# Autodesk Inventor assembly: робот
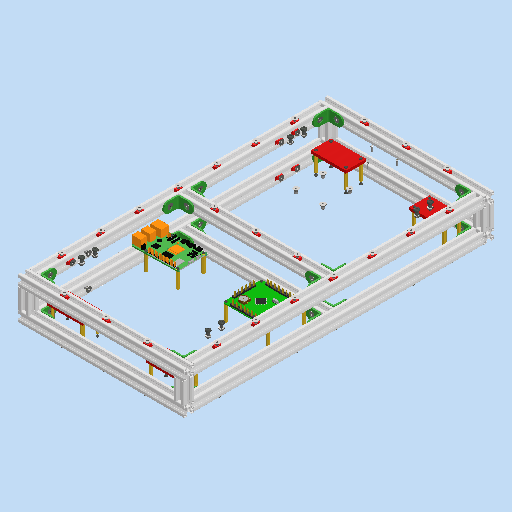
[picture p0: Inventor's stored thumbnail of the model, 512x512]
Saved by Autodesk Inventor 2025 (Build 290162000, 162)
## iProperties
Created: 2025-02-17
Part Number: робот
Document SubType Name: Assembly
Designer: volko
Mass: 11118.9 g
Surface Area: 27959 cm^2
Volume: 6182.29 cm^3
Density: 1.7985 g/cm^3
Author: volko
## Documents named in this file (62)
- C:\Users\volko\Desktop\диплом\Модели\детали\робот.iam
- C:\Users\volko\Desktop\диплом\Модели\детали\нижняя плита.ipt
- C:\Users\volko\Desktop\диплом\Модели\детали\правый привод.iam
- C:\Users\volko\Desktop\диплом\Модели\детали\левый привод.iam
- C:\Users\volko\Desktop\диплом\Модели\детали\рама.iam
- C:\Users\volko\Desktop\диплом\Модели\детали\верхняя плита.ipt
- C:\Users\volko\Desktop\диплом\Модели\детали\правый привод_MIR1.iam
- C:\Users\volko\Desktop\диплом\Модели\детали\левый привод_MIR1.iam
- C:\Users\volko\Desktop\диплом\Модели\детали\лидар.iam
- C:\Users\volko\Desktop\диплом\Модели\детали\сборка акб.iam
- C:\Users\volko\Desktop\диплом\Модели\детали\передний кожух.ipt
- C:\Users\volko\Desktop\диплом\Модели\детали\боковой кожух.ipt
- C:\Users\volko\Desktop\диплом\Модели\детали\гайка T-паза m5.ipt
- гайка T-паза m5.ipt
- C:\Users\volko\Desktop\диплом\Модели\детали\гайка T-паза m5_MIR.ipt
- C:\Users\volko\Desktop\диплом\Модели\детали\гайка T-паза m5_MIR_MIR.ipt
- C:\Users\volko\Desktop\диплом\Модели\детали\гайка T-паза m5_MIR1.ipt
- C:\Users\volko\Desktop\диплом\Модели\детали\гайка T-паза m5_MIR2.ipt
- C:\Users\volko\Desktop\диплом\Модели\детали\гайка T-паза m5_MIR_MIR1.ipt
- C:\Users\volko\Desktop\диплом\Модели\детали\лоток для маркеров.ipt
- C:\Users\volko\Desktop\диплом\Модели\детали\стандартные изделия\ru-RU\ISO 1580\ISO 1580 - M2 x 8_.ipt
- C:\Users\volko\Desktop\диплом\Модели\детали\сборка драйверов.iam
- C:\Users\volko\Desktop\диплом\Модели\детали\стандартные изделия\ru-RU\ISO 7045  H\ISO 7045 - M2,5 x 8_ - 4.8 - H - ISO.ipt
- C:\Users\volko\Desktop\диплом\Модели\детали\сборка драйверов_MIR2.iam
- C:\Users\volko\Desktop\диплом\Модели\детали\сборка драйверов_MIR3.iam
- C:\Users\volko\Desktop\диплом\Модели\детали\сборка драйверов_MIR2_MIR.iam
- C:\Users\volko\Desktop\диплом\Модели\детали\сборка raspberry pi.iam
- C:\Users\volko\Desktop\диплом\Модели\детали\сборка микроконтроллера.iam
- C:\Users\volko\Desktop\диплом\Модели\детали\стандартные изделия\ru-RU\DIN 7991(2)\DIN 7991 - M5x8.ipt
- C:\Users\volko\Desktop\диплом\Модели\детали\стандартные изделия\ru-RU\ISO 4035(2)\ISO 4035 - M5 - ISO.ipt
- C:\Users\volko\Desktop\диплом\Модели\детали\стандартные изделия\ru-RU\ISO 7380-1\ISO 7380-1 - M5 x 12.ipt
- C:\Users\volko\Desktop\диплом\Модели\детали\скоба.ipt
- C:\Users\volko\Desktop\диплом\Модели\детали\скоба_MIR.ipt
- C:\Users\volko\Desktop\диплом\Модели\детали\гайка T-паза m5_MIR_MIR1_MIR.ipt
- C:\Users\volko\Desktop\диплом\Модели\детали\скоба_MIR1.ipt
- C:\Users\volko\Desktop\диплом\Модели\детали\гайка T-паза m5_MIR_MIR1_MIR1.ipt
- C:\Users\volko\Desktop\диплом\Модели\детали\скоба_MIR_MIR.ipt
- C:\Users\volko\Desktop\диплом\Модели\детали\гайка T-паза m5_MIR_MIR1_MIR_MIR.ipt
- C:\Users\volko\Desktop\диплом\Модели\детали\скоба_MIR_MIR_MIR.ipt
- C:\Users\volko\Desktop\диплом\Модели\детали\гайка T-паза m5_MIR_MIR1_MIR_MIR_MIR.ipt
- C:\Users\volko\Desktop\диплом\Модели\детали\гайка T-паза m5_MIR_MIR1_MIR1_MIR.ipt
- C:\Users\volko\Desktop\диплом\Модели\детали\скоба_MIR1_MIR.ipt
- C:\Users\volko\Desktop\диплом\Модели\детали\скоба_MIR_MIR_MIR_MIR.ipt
- C:\Users\volko\Desktop\диплом\Модели\детали\гайка T-паза m5_MIR_MIR1_MIR_MIR_MIR_MIR.ipt
- C:\Users\volko\Desktop\диплом\Модели\детали\гайка T-паза m5_MIR_MIR1_MIR1_MIR_MIR.ipt
- C:\Users\volko\Desktop\диплом\Модели\детали\скоба_MIR1_MIR_MIR.ipt
- C:\Users\volko\Desktop\диплом\Модели\детали\скоба_MIR1_MIR_MIR_MIR.ipt
- C:\Users\volko\Desktop\диплом\Модели\детали\гайка T-паза m5_MIR_MIR1_MIR1_MIR_MIR_MIR.ipt
- C:\Users\volko\Desktop\диплом\Модели\детали\гайка T-паза m5_MIR_MIR1_MIR_MIR_MIR_MIR_MIR.ipt
- C:\Users\volko\Desktop\диплом\Модели\детали\скоба_MIR_MIR_MIR_MIR_MIR.ipt
- C:\Users\volko\Desktop\диплом\Модели\детали\скоба_MIR1_MIR_MIR1.ipt
- C:\Users\volko\Desktop\диплом\Модели\детали\гайка T-паза m5_MIR_MIR1_MIR1_MIR_MIR1.ipt
- C:\Users\volko\Desktop\диплом\Модели\детали\гайка T-паза m5_MIR_MIR1_MIR_MIR_MIR_MIR1.ipt
- C:\Users\volko\Desktop\диплом\Модели\детали\скоба_MIR_MIR_MIR_MIR1.ipt
- C:\Users\volko\Desktop\диплом\Модели\детали\скоба_MIR_MIR_MIR1.ipt
- C:\Users\volko\Desktop\диплом\Модели\детали\гайка T-паза m5_MIR_MIR1_MIR_MIR_MIR1.ipt
- C:\Users\volko\Desktop\диплом\Модели\детали\гайка T-паза m5_MIR_MIR1_MIR1_MIR1.ipt
- C:\Users\volko\Desktop\диплом\Модели\детали\скоба_MIR1_MIR1.ipt
- C:\Users\volko\Desktop\диплом\Модели\детали\гайка T-паза m5_MIR_MIR1_MIR_MIR2.ipt
- C:\Users\volko\Desktop\диплом\Модели\детали\скоба_MIR_MIR2.ipt
- C:\Users\volko\Desktop\диплом\Модели\детали\скоба_MIR4.ipt
- C:\Users\volko\Desktop\диплом\Модели\детали\гайка T-паза m5_MIR_MIR1_MIR3.ipt
## Components (261 placed, 60 different names)
1. рама:1 [sub-assembly] — Совмещение:1, Совмещение:3, Совмещение:4, Совмещение:12, Совмещение:13, Совмещение:15, Совмещение:16, Совмещение:18, Совмещение:19, Совмещение:20, Заподлицо:19, Заподлицо:20, Совмещение:23, Заподлицо:22, Совмещение:25, Совмещение:26, Совмещение:27, Совмещение:28, Совмещение:29, Совмещение:32, Совмещение:38, Угол:2, Совмещение:40, Угол:3, Заподлицо:60, Совмещение:88, Совмещение:89, Заподлицо:69
2. правый привод:1 [sub-assembly] — Совмещение:11, Заподлицо:10, Совмещение:12, Совмещение:80, Совмещение:81
3. левый привод:1 [sub-assembly] — Совмещение:3, Совмещение:4, Заподлицо:2, Совмещение:11, Заподлицо:10, Совмещение:13
4. правый привод_MIR1:1 [sub-assembly] — Заподлицо:12, Совмещение:14, Совмещение:19, Совмещение:21
5. левый привод_MIR1:1 [sub-assembly] — Заподлицо:12, Совмещение:14, Совмещение:15, Совмещение:20, Совмещение:33, Совмещение:34, Совмещение:35, Совмещение:36, Совмещение:37
6. нижняя плита:1 — Заподлицо:14, Совмещение:16, Заподлицо:21, Совмещение:25, Заподлицо:27, Заподлицо:30, Заподлицо:31, Заподлицо:32, Совмещение:41, Совмещение:42, Совмещение:43, Совмещение:44, Заподлицо:35, Совмещение:58, Совмещение:59, Совмещение:60, Совмещение:61, Совмещение:62, Совмещение:63, Совмещение:64, Совмещение:65, Совмещение:66, Совмещение:67, Совмещение:72, Совмещение:73
7. верхняя плита:1 — Совмещение:17, Совмещение:18, Заподлицо:22, Совмещение:24, Совмещение:48, Совмещение:49, Совмещение:50, Совмещение:51, Заподлицо:37, Заподлицо:38, Заподлицо:39, Заподлицо:40, Заподлицо:41, Заподлицо:42, Заподлицо:43, Заподлицо:44, Заподлицо:45, Заподлицо:46, Заподлицо:47, Заподлицо:48, Заподлицо:49, Заподлицо:50, Заподлицо:51, Заподлицо:52, Заподлицо:53, Заподлицо:54, Заподлицо:55, Заподлицо:56, Заподлицо:57, Заподлицо:58, Заподлицо:59, Совмещение:74, Совмещение:75, Совмещение:76, Совмещение:77
8. лидар:1 [sub-assembly] — Совмещение:24, Заподлицо:26, Совмещение:51, Совмещение:52, Совмещение:53, Совмещение:54, Совмещение:55, Совмещение:56, Совмещение:57
9. сборка акб:1 [sub-assembly] — Заподлицо:21, Совмещение:22, Совмещение:23
10. передний кожух:1 — Совмещение:26, Заподлицо:27, Заподлицо:33
11. передний кожух:2 — Совмещение:27, Заподлицо:30, Заподлицо:34
12. боковой кожух:1 — Совмещение:28, Заподлицо:31, Совмещение:30
13. боковой кожух:2 — Совмещение:29, Заподлицо:32, Совмещение:31
14. лоток для маркеров:1 — Совмещение:47, Совмещение:48, Совмещение:49, Заподлицо:36
15. сборка драйверов:1 [sub-assembly] — Совмещение:58, Совмещение:59, Совмещение:68
16. сборка драйверов_MIR2:1 [sub-assembly] — Совмещение:69
17. сборка драйверов_MIR3:1 [sub-assembly] — Совмещение:70
18. сборка драйверов_MIR2_MIR:1 [sub-assembly] — Совмещение:71
19. сборка raspberry pi:1 [sub-assembly] — Совмещение:72
20. сборка микроконтроллера:1 [sub-assembly] — Совмещение:73
21. скоба_MIR1_MIR_MIR_MIR:1 — Совмещение:180, Совмещение:181, Угол:38, Совмещение:182, Совмещение:183, Угол:39, Заподлицо:96, Заподлицо:97
22. гайка T-паза m5_MIR_MIR1_MIR1_MIR_MIR_MIR:1 — Совмещение:180, Совмещение:181, Угол:38
23. гайка T-паза m5_MIR_MIR1_MIR1_MIR_MIR_MIR:2 — Совмещение:182, Совмещение:183, Угол:39
24. DIN 7991 M5x8:95 — Заподлицо:96
25. DIN 7991 M5x8:96 — Заподлицо:97
26. гайка T-паза m5_MIR_MIR1_MIR_MIR_MIR_MIR_MIR:1 — Угол:37, Совмещение:178, Совмещение:179
27. гайка T-паза m5_MIR_MIR1_MIR_MIR_MIR_MIR_MIR:2 — Угол:36, Совмещение:175, Совмещение:176, Совмещение:177
28. скоба_MIR_MIR_MIR_MIR_MIR:1 — Заподлицо:94, Совмещение:174, Заподлицо:95, Угол:36, Совмещение:175, Совмещение:176, Угол:37, Совмещение:178, Совмещение:179
29. DIN 7991 M5x8:97 — Заподлицо:95, Совмещение:177
30. DIN 7991 M5x8:98 — Заподлицо:94, Совмещение:174
31. скоба_MIR1_MIR_MIR1:1 — Заподлицо:92, Заподлицо:93, Угол:34, Совмещение:170, Совмещение:171, Угол:35, Совмещение:172, Совмещение:173
32. гайка T-паза m5_MIR_MIR1_MIR1_MIR_MIR1:1 — Угол:35, Совмещение:172, Совмещение:173
33. гайка T-паза m5_MIR_MIR1_MIR1_MIR_MIR1:2 — Угол:34, Совмещение:170, Совмещение:171
34. DIN 7991 M5x8:99 — Заподлицо:93
35. DIN 7991 M5x8:100 — Заподлицо:92
36. гайка T-паза m5_MIR_MIR1_MIR_MIR_MIR_MIR1:1 — Совмещение:168, Совмещение:169, Угол:33
37. гайка T-паза m5_MIR_MIR1_MIR_MIR_MIR_MIR1:2 — Совмещение:165, Совмещение:166, Совмещение:167, Угол:32
38. скоба_MIR_MIR_MIR_MIR1:1 — Заподлицо:90, Совмещение:164, Заподлицо:91, Совмещение:166, Совмещение:167, Угол:32, Совмещение:168, Совмещение:169, Угол:33
39. DIN 7991 M5x8:101 — Заподлицо:90, Совмещение:165
40. DIN 7991 M5x8:102 — Совмещение:164, Заподлицо:91
41. скоба_MIR_MIR_MIR1:1 — Угол:30, Совмещение:158, Совмещение:159, Угол:31, Совмещение:160, Совмещение:161, Заподлицо:88, Совмещение:162, Заподлицо:89
42. DIN 7991 M5x8:103 — Совмещение:163, Заподлицо:89
43. DIN 7991 M5x8:104 — Заподлицо:88, Совмещение:162
44. гайка T-паза m5_MIR_MIR1_MIR_MIR_MIR1:1 — Угол:31, Совмещение:160, Совмещение:161, Совмещение:163
45. гайка T-паза m5_MIR_MIR1_MIR_MIR_MIR1:2 — Угол:30, Совмещение:158, Совмещение:159
46. DIN 7991 M5x8:105 — Заподлицо:87
47. DIN 7991 M5x8:106 — Заподлицо:86
48. гайка T-паза m5_MIR_MIR1_MIR1_MIR1:1 — Совмещение:156, Совмещение:157, Угол:29
49. гайка T-паза m5_MIR_MIR1_MIR1_MIR1:2 — Совмещение:154, Совмещение:155, Угол:28
50. скоба_MIR1_MIR1:1 — Совмещение:154, Совмещение:155, Угол:28, Совмещение:156, Совмещение:157, Угол:29, Заподлицо:86, Заподлицо:87
51. DIN 7991 M5x8:107 — Заподлицо:85
52. DIN 7991 M5x8:108 — Заподлицо:84
53. гайка T-паза m5_MIR_MIR1_MIR_MIR2:1 — Совмещение:152, Совмещение:153, Угол:27
54. гайка T-паза m5_MIR_MIR1_MIR_MIR2:2 — Совмещение:150, Совмещение:151, Угол:26
55. скоба_MIR_MIR2:1 — Совмещение:150, Совмещение:151, Угол:26, Совмещение:152, Совмещение:153, Угол:27, Заподлицо:84, Заподлицо:85
56. скоба_MIR4:1 — Угол:24, Совмещение:144, Совмещение:145, Угол:25, Совмещение:146, Совмещение:147, Заподлицо:82, Совмещение:148, Заподлицо:83
57. гайка T-паза m5_MIR_MIR1_MIR3:1 — Угол:24, Совмещение:144, Совмещение:145
58. гайка T-паза m5_MIR_MIR1_MIR3:2 — Угол:25, Совмещение:146, Совмещение:147, Совмещение:149
59. DIN 7991 M5x8:109 — Заподлицо:82, Совмещение:148
60. DIN 7991 M5x8:110 — Совмещение:149, Заподлицо:83
61. ISO 7380-1 M5 x 12:8 — Совмещение:87
62. ISO 7380-1 M5 x 12:7 — Совмещение:86
63. ISO 4035 M5:8 — Совмещение:87
64. ISO 4035 M5:7 — Совмещение:86
65. ISO 7380-1 M5 x 12:6 — Совмещение:85
66. ISO 7380-1 M5 x 12:5 — Совмещение:84
67. ISO 4035 M5:6 — Совмещение:85
68. ISO 4035 M5:5 — Совмещение:84
69. ISO 7380-1 M5 x 12:4 — Совмещение:83
70. ISO 7380-1 M5 x 12:3 — Совмещение:82
71. ISO 4035 M5:4 — Совмещение:83
72. ISO 4035 M5:3 — Совмещение:82
73. ISO 7380-1 M5 x 12:2 — Совмещение:75, Совмещение:77, Совмещение:79
74. ISO 7380-1 M5 x 12:1 — Совмещение:74, Совмещение:76, Совмещение:78
75. ISO 4035 M5:2 — Совмещение:79, Совмещение:81
76. ISO 4035 M5:1 — Совмещение:78, Совмещение:80
77. DIN 7991 M5x8:74
78. DIN 7991 M5x8:73
79. DIN 7991 M5x8:72
80. DIN 7991 M5x8:71
81. DIN 7991 M5x8:78
82. DIN 7991 M5x8:77
83. DIN 7991 M5x8:76
84. DIN 7991 M5x8:75
85. DIN 7991 M5x8:70
86. DIN 7991 M5x8:69
87. DIN 7991 M5x8:68
88. DIN 7991 M5x8:67
89. ISO 7045 H M2,5 x 8 - 4.8 - H:5
90. ISO 7045 H M2,5 x 8 - 4.8 - H:6
91. ISO 7045 H M2,5 x 8 - 4.8 - H:7
92. ISO 7045 H M2,5 x 8 - 4.8 - H:8 — Совмещение:69
93. ISO 7045 H M2,5 x 8 - 4.8 - H:9
94. ISO 7045 H M2,5 x 8 - 4.8 - H:10
95. ISO 7045 H M2,5 x 8 - 4.8 - H:11
96. ISO 7045 H M2,5 x 8 - 4.8 - H:12 — Совмещение:70
97. ISO 7045 H M2,5 x 8 - 4.8 - H:13
98. ISO 7045 H M2,5 x 8 - 4.8 - H:14
99. ISO 7045 H M2,5 x 8 - 4.8 - H:15
100. ISO 7045 H M2,5 x 8 - 4.8 - H:16 — Совмещение:71
101. ISO 7045 H M2,5 x 8 - 4.8 - H:1 — Совмещение:60, Совмещение:66
102. ISO 7045 H M2,5 x 8 - 4.8 - H:2 — Совмещение:63, Совмещение:65
103. ISO 7045 H M2,5 x 8 - 4.8 - H:3 — Совмещение:62, Совмещение:64
104. ISO 7045 H M2,5 x 8 - 4.8 - H:4 — Совмещение:61, Совмещение:67, Совмещение:68
105. ISO 1580 M2 x 8:3 — Совмещение:54, Совмещение:55
106. ISO 1580 M2 x 8:2 — Совмещение:53, Совмещение:57
107. ISO 1580 M2 x 8:1 — Совмещение:52, Совмещение:56
108. гайка T-паза m5_MIR_MIR1:10
109. гайка T-паза m5_MIR_MIR1:11
110. гайка T-паза m5_MIR_MIR1:13
111. гайка T-паза m5_MIR_MIR1:12
112. гайка T-паза m5_MIR_MIR1:14
113. DIN 7991 M5x8:2 — Заподлицо:37
114. DIN 7991 M5x8:3 — Заподлицо:56
115. DIN 7991 M5x8:4 — Заподлицо:47
116. DIN 7991 M5x8:5 — Заподлицо:38
117. DIN 7991 M5x8:6 — Заподлицо:55
118. DIN 7991 M5x8:7 — Заподлицо:48
119. DIN 7991 M5x8:8 — Заподлицо:40
120. DIN 7991 M5x8:9 — Заподлицо:54
121. DIN 7991 M5x8:10 — Заподлицо:49
122. DIN 7991 M5x8:11 — Совмещение:46, Заподлицо:39
123. DIN 7991 M5x8:12 — Заподлицо:59
124. DIN 7991 M5x8:13 — Заподлицо:41
125. DIN 7991 M5x8:14 — Заподлицо:58
126. DIN 7991 M5x8:15 — Заподлицо:42
127. DIN 7991 M5x8:16 — Заподлицо:57
128. DIN 7991 M5x8:17 — Заподлицо:43
129. DIN 7991 M5x8:18 — Заподлицо:53
130. DIN 7991 M5x8:19 — Заподлицо:44
131. DIN 7991 M5x8:20 — Заподлицо:52
132. DIN 7991 M5x8:21 — Заподлицо:45
133. DIN 7991 M5x8:22 — Заподлицо:51
134. DIN 7991 M5x8:23 — Заподлицо:46
135. DIN 7991 M5x8:24 — Заподлицо:50
136. гайка T-паза m5_MIR2:7
137. гайка T-паза m5_MIR2:6
138. гайка T-паза m5_MIR2:5
139. гайка T-паза m5_MIR2:2
140. гайка T-паза m5_MIR2:1
141. гайка T-паза m5_MIR2:4
142. гайка T-паза m5_MIR2:3
143. гайка T-паза m5_MIR2:8
144. гайка T-паза m5_MIR2:9
145. гайка T-паза m5_MIR_MIR1:1 — Совмещение:46
146. гайка T-паза m5_MIR_MIR1:2
147. гайка T-паза m5_MIR_MIR1:3
148. гайка T-паза m5_MIR_MIR1:4
149. гайка T-паза m5_MIR_MIR1:6
150. гайка T-паза m5_MIR_MIR1:5
151. гайка T-паза m5_MIR_MIR1:7
152. гайка T-паза m5_MIR_MIR1:8
153. гайка T-паза m5_MIR_MIR1:9
154. гайка T-паза m5_MIR1:4
155. гайка T-паза m5_MIR1:3
156. гайка T-паза m5_MIR1:2
157. гайка T-паза m5_MIR1:1
158. гайка T-паза m5_MIR_MIR:4
159. гайка T-паза m5_MIR_MIR:3
160. гайка T-паза m5_MIR_MIR:2
161. гайка T-паза m5_MIR_MIR:1
162. гайка T-паза m5_MIR:4
163. гайка T-паза m5_MIR:3
164. гайка T-паза m5_MIR:2
165. гайка T-паза m5_MIR:1
166. DIN 7991 M5x8:37 — Совмещение:34
167. DIN 7991 M5x8:38 — Совмещение:35
168. DIN 7991 M5x8:39 — Совмещение:36
169. DIN 7991 M5x8:1 — Совмещение:37
170. скоба_MIR1_MIR_MIR:1 — Заподлицо:80, Заподлицо:81, Угол:22, Совмещение:140, Совмещение:141, Угол:23, Совмещение:142, Совмещение:143
171. гайка T-паза m5_MIR_MIR1_MIR1_MIR_MIR:2 — Угол:23, Совмещение:142, Совмещение:143
172. гайка T-паза m5_MIR_MIR1_MIR1_MIR_MIR:1 — Угол:22, Совмещение:140, Совмещение:141
173. DIN 7991 M5x8:94 — Заподлицо:81
174. DIN 7991 M5x8:93 — Заподлицо:80
175. гайка T-паза m5_MIR_MIR1_MIR_MIR_MIR_MIR:2 — Совмещение:138, Совмещение:139, Угол:21
176. гайка T-паза m5_MIR_MIR1_MIR_MIR_MIR_MIR:1 — Совмещение:135, Совмещение:136, Совмещение:137, Угол:20
177. скоба_MIR_MIR_MIR_MIR:1 — Заподлицо:78, Совмещение:134, Заподлицо:79, Совмещение:136, Совмещение:137, Угол:20, Совмещение:138, Совмещение:139, Угол:21
178. DIN 7991 M5x8:92 — Заподлицо:78, Совмещение:135
179. DIN 7991 M5x8:91 — Совмещение:134, Заподлицо:79
180. скоба_MIR1_MIR:1 — Совмещение:124, Совмещение:125, Угол:16, Совмещение:126, Совмещение:127, Угол:17, Заподлицо:74, Заподлицо:75
181. гайка T-паза m5_MIR_MIR1_MIR1_MIR:2 — Совмещение:124, Совмещение:125, Угол:16
182. гайка T-паза m5_MIR_MIR1_MIR1_MIR:1 — Совмещение:126, Совмещение:127, Угол:17
183. DIN 7991 M5x8:90 — Заподлицо:74
184. DIN 7991 M5x8:89 — Заподлицо:75
185. гайка T-паза m5_MIR_MIR1_MIR_MIR_MIR:2 — Угол:18, Совмещение:128, Совмещение:129
186. гайка T-паза m5_MIR_MIR1_MIR_MIR_MIR:1 — Угол:19, Совмещение:130, Совмещение:131, Совмещение:133
187. скоба_MIR_MIR_MIR:1 — Угол:18, Совмещение:128, Совмещение:129, Угол:19, Совмещение:130, Совмещение:131, Заподлицо:76, Совмещение:132, Заподлицо:77
188. DIN 7991 M5x8:87 — Совмещение:133, Заподлицо:77
189. DIN 7991 M5x8:88 — Заподлицо:76, Совмещение:132
190. скоба_MIR_MIR:1 — Совмещение:108, Совмещение:109, Угол:10, Совмещение:110, Совмещение:111, Угол:11, Совмещение:112, Заподлицо:67, Заподлицо:68
191. DIN 7991 M5x8:86 — Заподлицо:68, Совмещение:113
192. DIN 7991 M5x8:85 — Совмещение:112, Заподлицо:67
193. гайка T-паза m5_MIR_MIR1_MIR_MIR:2 — Совмещение:110, Совмещение:111, Угол:11, Совмещение:113
194. гайка T-паза m5_MIR_MIR1_MIR_MIR:1 — Совмещение:108, Совмещение:109, Угол:10
195. DIN 7991 M5x8:84 — Заподлицо:66
196. DIN 7991 M5x8:83 — Заподлицо:65
197. гайка T-паза m5_MIR_MIR1_MIR1:2 — Угол:9, Совмещение:104, Совмещение:105
198. гайка T-паза m5_MIR_MIR1_MIR1:1 — Угол:8, Совмещение:102, Совмещение:103
199. скоба_MIR1:1 — Угол:8, Совмещение:102, Совмещение:103, Угол:9, Совмещение:104, Совмещение:105, Заподлицо:65, Заподлицо:66
200. DIN 7991 M5x8:82 — Заподлицо:64
201. DIN 7991 M5x8:81 — Заподлицо:63
202. гайка T-паза m5_MIR_MIR1_MIR:2 — Угол:7, Совмещение:98, Совмещение:99
203. гайка T-паза m5_MIR_MIR1_MIR:1 — Угол:6, Совмещение:96, Совмещение:97
204. скоба_MIR:1 — Угол:6, Совмещение:96, Совмещение:97, Угол:7, Совмещение:98, Совмещение:99, Заподлицо:63, Заподлицо:64
205. скоба:1 — Заподлицо:60, Совмещение:88, Совмещение:89, Совмещение:90, Совмещение:91, Совмещение:92, Совмещение:93, Угол:4, Угол:5, Совмещение:94, Заподлицо:61, Заподлицо:62
206. гайка T-паза m5_MIR_MIR1:15 — Совмещение:90, Совмещение:92, Угол:4
207. гайка T-паза m5_MIR_MIR1:16 — Совмещение:91, Совмещение:93, Угол:5, Совмещение:95
208. DIN 7991 M5x8:79 — Совмещение:94, Заподлицо:61
209. DIN 7991 M5x8:80 — Заподлицо:62, Совмещение:95
210. DIN 7991 M5x8:63 — Совмещение:50, Заподлицо:36
211. DIN 7991 M5x8:64
212. DIN 7991 M5x8:65
213. DIN 7991 M5x8:66
214. DIN 7991 M5x8:49 — Совмещение:45, Заподлицо:35
215. DIN 7991 M5x8:50
216. DIN 7991 M5x8:51
217. DIN 7991 M5x8:52
218. DIN 7991 M5x8:53
219. DIN 7991 M5x8:54
220. DIN 7991 M5x8:55
221. DIN 7991 M5x8:56
222. DIN 7991 M5x8:57
223. DIN 7991 M5x8:58
224. DIN 7991 M5x8:59
225. DIN 7991 M5x8:60
226. DIN 7991 M5x8:61
227. DIN 7991 M5x8:62
228. гайка T-паза m5_MIR:5 — Совмещение:40, Угол:3, Совмещение:42, Совмещение:45
229. гайка T-паза m5_MIR:6
230. гайка T-паза m5_MIR:7
231. гайка T-паза m5_MIR:8
232. гайка T-паза m5_MIR:9
233. гайка T-паза m5_MIR:10
234. гайка T-паза m5_MIR:11
235. гайка T-паза m5_MIR:12
236. гайка T-паза m5_MIR:13
237. гайка T-паза m5_MIR:14
238. гайка T-паза m5_MIR:15
239. гайка T-паза m5_MIR:16
240. гайка T-паза m5_MIR:17
241. гайка T-паза m5_MIR:18
242. DIN 7991 M5x8:40 — Совмещение:43, Совмещение:44
243. DIN 7991 M5x8:41
244. DIN 7991 M5x8:42
245. DIN 7991 M5x8:43
246. DIN 7991 M5x8:44
247. DIN 7991 M5x8:45
248. DIN 7991 M5x8:46
249. DIN 7991 M5x8:47
250. DIN 7991 M5x8:48
251. гайка T-паза m5:5 — Совмещение:38, Угол:2, Совмещение:41
252. гайка T-паза m5:6
253. гайка T-паза m5:7
254. гайка T-паза m5:8
255. гайка T-паза m5:9
256. гайка T-паза m5:10
257. гайка T-паза m5:11
258. гайка T-паза m5:12
259. гайка T-паза m5:13
260. гайка T-паза m5:1 — Совмещение:32, Совмещение:33, Угол:1
261. гайка T-паза m5:2
## Component patterns: (4 elements, first: DIN 7991 M5x8:63), (14 elements, first: DIN 7991 M5x8:49), (14 elements, first: гайка T-паза m5_MIR:5), (9 elements, first: DIN 7991 M5x8:40), (9 elements, first: гайка T-паза m5:5), (2 elements, first: гайка T-паза m5:1)
## Relationships (271: Mate 161, Flush 75, Angle 35)
- Совмещение:1 [Mate]: рама:1
- Совмещение:3 [Mate]: рама:1 ↔ левый привод:1
- Совмещение:4 [Mate]: рама:1 ↔ левый привод:1
- Заподлицо:2 [Flush]: левый привод:1
- Совмещение:11 [Mate]: правый привод:1 ↔ левый привод:1
- Заподлицо:10 [Flush]: правый привод:1 ↔ левый привод:1
- Совмещение:12 [Mate]: рама:1 ↔ правый привод:1
- Совмещение:13 [Mate] (50 mm): рама:1 ↔ левый привод:1
- Заподлицо:12 [Flush]: правый привод_MIR1:1 ↔ левый привод_MIR1:1
- Совмещение:14 [Mate]: правый привод_MIR1:1 ↔ левый привод_MIR1:1
- Совмещение:15 [Mate] (50 mm): рама:1 ↔ левый привод_MIR1:1
- Заподлицо:14 [Flush]: нижняя плита:1
- Совмещение:16 [Mate]: рама:1 ↔ нижняя плита:1
- Совмещение:17 [Mate]: верхняя плита:1
- Совмещение:18 [Mate]: рама:1 ↔ верхняя плита:1
- Совмещение:19 [Mate]: рама:1 ↔ правый привод_MIR1:1
- Совмещение:20 [Mate]: рама:1 ↔ левый привод_MIR1:1
- Заподлицо:18 [Flush]
- Заподлицо:19 [Flush]: рама:1
- Заподлицо:20 [Flush]: рама:1
- Совмещение:21 [Mate]: правый привод_MIR1:1
- Заподлицо:21 [Flush]: нижняя плита:1 ↔ сборка акб:1
- Совмещение:22 [Mate]: сборка акб:1
- Совмещение:23 [Mate] (10 mm): рама:1 ↔ сборка акб:1
- Заподлицо:22 [Flush]: рама:1 ↔ верхняя плита:1
- Совмещение:24 [Mate]: верхняя плита:1 ↔ лидар:1
- Заподлицо:26 [Flush]: лидар:1
- Совмещение:25 [Mate]: рама:1 ↔ нижняя плита:1
- Совмещение:26 [Mate]: рама:1 ↔ передний кожух:1
- Заподлицо:27 [Flush]: нижняя плита:1 ↔ передний кожух:1
- Совмещение:27 [Mate]: рама:1 ↔ передний кожух:2
- Заподлицо:30 [Flush]: нижняя плита:1 ↔ передний кожух:2
- Совмещение:28 [Mate]: рама:1 ↔ боковой кожух:1
- Совмещение:29 [Mate]: рама:1 ↔ боковой кожух:2
- Заподлицо:31 [Flush]: нижняя плита:1 ↔ боковой кожух:1
- Заподлицо:32 [Flush]: нижняя плита:1 ↔ боковой кожух:2
- Заподлицо:33 [Flush]: передний кожух:1
- Заподлицо:34 [Flush]: передний кожух:2
- Совмещение:30 [Mate]: боковой кожух:1
- Совмещение:31 [Mate]: боковой кожух:2
- Совмещение:32 [Mate]: рама:1 ↔ гайка T-паза m5:1
- Совмещение:33 [Mate]: левый привод_MIR1:1 ↔ гайка T-паза m5:1
- Угол:1 [Angle] (0 deg): гайка T-паза m5:1
- Совмещение:34 [Mate]: левый привод_MIR1:1 ↔ DIN 7991 M5x8:37
- Совмещение:35 [Mate]: левый привод_MIR1:1 ↔ DIN 7991 M5x8:38
- Совмещение:36 [Mate]: левый привод_MIR1:1 ↔ DIN 7991 M5x8:39
- Совмещение:37 [Mate]: левый привод_MIR1:1 ↔ DIN 7991 M5x8:1
- Совмещение:38 [Mate]: рама:1 ↔ гайка T-паза m5:5
- Угол:2 [Angle] (0 deg): рама:1 ↔ гайка T-паза m5:5
- Совмещение:40 [Mate]: рама:1 ↔ гайка T-паза m5_MIR:5
- Угол:3 [Angle] (0 deg): рама:1 ↔ гайка T-паза m5_MIR:5
- Совмещение:41 [Mate]: нижняя плита:1 ↔ гайка T-паза m5:5
- Совмещение:42 [Mate]: нижняя плита:1 ↔ гайка T-паза m5_MIR:5
- Совмещение:43 [Mate]: нижняя плита:1 ↔ DIN 7991 M5x8:40
- Совмещение:44 [Mate]: нижняя плита:1 ↔ DIN 7991 M5x8:40
- Совмещение:45 [Mate]: DIN 7991 M5x8:49 ↔ гайка T-паза m5_MIR:5
- Заподлицо:35 [Flush]: нижняя плита:1 ↔ DIN 7991 M5x8:49
- Совмещение:46 [Mate]: DIN 7991 M5x8:11 ↔ гайка T-паза m5_MIR_MIR1:1
- Совмещение:47 [Mate]: лоток для маркеров:1
- Совмещение:48 [Mate]: верхняя плита:1 ↔ лоток для маркеров:1
- Совмещение:49 [Mate]: верхняя плита:1 ↔ лоток для маркеров:1
- Совмещение:50 [Mate]: верхняя плита:1 ↔ DIN 7991 M5x8:63
- Заподлицо:36 [Flush]: лоток для маркеров:1 ↔ DIN 7991 M5x8:63
- Совмещение:51 [Mate]: верхняя плита:1 ↔ лидар:1
- Совмещение:52 [Mate]: лидар:1 ↔ ISO 1580 M2 x 8:1
- Совмещение:53 [Mate]: лидар:1 ↔ ISO 1580 M2 x 8:2
- Совмещение:54 [Mate]: лидар:1 ↔ ISO 1580 M2 x 8:3
- Совмещение:55 [Mate]: лидар:1 ↔ ISO 1580 M2 x 8:3
- Совмещение:56 [Mate]: лидар:1 ↔ ISO 1580 M2 x 8:1
- Совмещение:57 [Mate]: лидар:1 ↔ ISO 1580 M2 x 8:2
- Заподлицо:37 [Flush]: верхняя плита:1 ↔ DIN 7991 M5x8:2
- Заподлицо:38 [Flush]: верхняя плита:1 ↔ DIN 7991 M5x8:5
- Заподлицо:39 [Flush]: верхняя плита:1 ↔ DIN 7991 M5x8:11
- Заподлицо:40 [Flush]: верхняя плита:1 ↔ DIN 7991 M5x8:8
- Заподлицо:41 [Flush]: верхняя плита:1 ↔ DIN 7991 M5x8:13
- Заподлицо:42 [Flush]: верхняя плита:1 ↔ DIN 7991 M5x8:15
- Заподлицо:43 [Flush]: верхняя плита:1 ↔ DIN 7991 M5x8:17
- Заподлицо:44 [Flush]: верхняя плита:1 ↔ DIN 7991 M5x8:19
- Заподлицо:45 [Flush]: верхняя плита:1 ↔ DIN 7991 M5x8:21
- Заподлицо:46 [Flush]: верхняя плита:1 ↔ DIN 7991 M5x8:23
- Заподлицо:47 [Flush]: верхняя плита:1 ↔ DIN 7991 M5x8:4
- Заподлицо:48 [Flush]: верхняя плита:1 ↔ DIN 7991 M5x8:7
- Заподлицо:49 [Flush]: верхняя плита:1 ↔ DIN 7991 M5x8:10
- Заподлицо:50 [Flush]: верхняя плита:1 ↔ DIN 7991 M5x8:24
- Заподлицо:51 [Flush]: верхняя плита:1 ↔ DIN 7991 M5x8:22
- Заподлицо:52 [Flush]: верхняя плита:1 ↔ DIN 7991 M5x8:20
- Заподлицо:53 [Flush]: верхняя плита:1 ↔ DIN 7991 M5x8:18
- Заподлицо:54 [Flush]: верхняя плита:1 ↔ DIN 7991 M5x8:9
- Заподлицо:55 [Flush]: верхняя плита:1 ↔ DIN 7991 M5x8:6
- Заподлицо:56 [Flush]: верхняя плита:1 ↔ DIN 7991 M5x8:3
- Заподлицо:57 [Flush]: верхняя плита:1 ↔ DIN 7991 M5x8:16
- Заподлицо:58 [Flush]: верхняя плита:1 ↔ DIN 7991 M5x8:14
- Заподлицо:59 [Flush]: верхняя плита:1 ↔ DIN 7991 M5x8:12
- Совмещение:58 [Mate]: нижняя плита:1 ↔ сборка драйверов:1
- Совмещение:59 [Mate]: нижняя плита:1 ↔ сборка драйверов:1
- Совмещение:60 [Mate]: нижняя плита:1 ↔ ISO 7045 H M2,5 x 8 - 4.8 - H:1
- Совмещение:61 [Mate]: нижняя плита:1 ↔ ISO 7045 H M2,5 x 8 - 4.8 - H:4
- Совмещение:62 [Mate]: нижняя плита:1 ↔ ISO 7045 H M2,5 x 8 - 4.8 - H:3
- Совмещение:63 [Mate]: нижняя плита:1 ↔ ISO 7045 H M2,5 x 8 - 4.8 - H:2
- Совмещение:64 [Mate]: нижняя плита:1 ↔ ISO 7045 H M2,5 x 8 - 4.8 - H:3
- Совмещение:65 [Mate]: нижняя плита:1 ↔ ISO 7045 H M2,5 x 8 - 4.8 - H:2
- Совмещение:66 [Mate]: нижняя плита:1 ↔ ISO 7045 H M2,5 x 8 - 4.8 - H:1
- Совмещение:67 [Mate]: нижняя плита:1 ↔ ISO 7045 H M2,5 x 8 - 4.8 - H:4
- Совмещение:68 [Mate]: сборка драйверов:1 ↔ ISO 7045 H M2,5 x 8 - 4.8 - H:4
- Совмещение:69 [Mate]: сборка драйверов_MIR2:1 ↔ ISO 7045 H M2,5 x 8 - 4.8 - H:8
- Совмещение:70 [Mate]: сборка драйверов_MIR3:1 ↔ ISO 7045 H M2,5 x 8 - 4.8 - H:12
- Совмещение:71 [Mate]: сборка драйверов_MIR2_MIR:1 ↔ ISO 7045 H M2,5 x 8 - 4.8 - H:16
- Совмещение:72 [Mate]: нижняя плита:1 ↔ сборка raspberry pi:1
- Совмещение:73 [Mate]: нижняя плита:1 ↔ сборка микроконтроллера:1
- Совмещение:74 [Mate]: верхняя плита:1 ↔ ISO 7380-1 M5 x 12:1
- Совмещение:75 [Mate]: верхняя плита:1 ↔ ISO 7380-1 M5 x 12:2
- Совмещение:76 [Mate]: верхняя плита:1 ↔ ISO 7380-1 M5 x 12:1
- Совмещение:77 [Mate]: верхняя плита:1 ↔ ISO 7380-1 M5 x 12:2
- Совмещение:78 [Mate]: ISO 7380-1 M5 x 12:1 ↔ ISO 4035 M5:1
- Совмещение:79 [Mate]: ISO 7380-1 M5 x 12:2 ↔ ISO 4035 M5:2
- Совмещение:80 [Mate]: правый привод:1 ↔ ISO 4035 M5:1
- Совмещение:81 [Mate]: правый привод:1 ↔ ISO 4035 M5:2
- Совмещение:82 [Mate]: ISO 7380-1 M5 x 12:3 ↔ ISO 4035 M5:3
- Совмещение:83 [Mate]: ISO 7380-1 M5 x 12:4 ↔ ISO 4035 M5:4
- Совмещение:84 [Mate]: ISO 7380-1 M5 x 12:5 ↔ ISO 4035 M5:5
- Совмещение:85 [Mate]: ISO 7380-1 M5 x 12:6 ↔ ISO 4035 M5:6
- Совмещение:86 [Mate]: ISO 7380-1 M5 x 12:7 ↔ ISO 4035 M5:7
- Совмещение:87 [Mate]: ISO 7380-1 M5 x 12:8 ↔ ISO 4035 M5:8
- Заподлицо:60 [Flush]: рама:1 ↔ скоба:1
- Совмещение:88 [Mate]: рама:1 ↔ скоба:1
- Совмещение:89 [Mate]: рама:1 ↔ скоба:1
- Совмещение:90 [Mate]: скоба:1 ↔ гайка T-паза m5_MIR_MIR1:15
- Совмещение:91 [Mate]: скоба:1 ↔ гайка T-паза m5_MIR_MIR1:16
- Совмещение:92 [Mate]: скоба:1 ↔ гайка T-паза m5_MIR_MIR1:15
- Совмещение:93 [Mate]: скоба:1 ↔ гайка T-паза m5_MIR_MIR1:16
- Угол:4 [Angle] (0 deg): скоба:1 ↔ гайка T-паза m5_MIR_MIR1:15
- Угол:5 [Angle] (0 deg): скоба:1 ↔ гайка T-паза m5_MIR_MIR1:16
- Совмещение:94 [Mate]: скоба:1 ↔ DIN 7991 M5x8:79
- Заподлицо:61 [Flush]: скоба:1 ↔ DIN 7991 M5x8:79
- Заподлицо:62 [Flush]: скоба:1 ↔ DIN 7991 M5x8:80
- Совмещение:95 [Mate]: гайка T-паза m5_MIR_MIR1:16 ↔ DIN 7991 M5x8:80
- Угол:6 [Angle] (0 deg): гайка T-паза m5_MIR_MIR1_MIR:1 ↔ скоба_MIR:1
- Совмещение:96 [Mate]: гайка T-паза m5_MIR_MIR1_MIR:1 ↔ скоба_MIR:1
- Совмещение:97 [Mate]: гайка T-паза m5_MIR_MIR1_MIR:1 ↔ скоба_MIR:1
- Угол:7 [Angle] (0 deg): гайка T-паза m5_MIR_MIR1_MIR:2 ↔ скоба_MIR:1
- Совмещение:98 [Mate]: гайка T-паза m5_MIR_MIR1_MIR:2 ↔ скоба_MIR:1
- Совмещение:99 [Mate]: гайка T-паза m5_MIR_MIR1_MIR:2 ↔ скоба_MIR:1
- Заподлицо:63 [Flush]: DIN 7991 M5x8:81 ↔ скоба_MIR:1
- Заподлицо:64 [Flush]: DIN 7991 M5x8:82 ↔ скоба_MIR:1
- Угол:8 [Angle] (0 deg): гайка T-паза m5_MIR_MIR1_MIR1:1 ↔ скоба_MIR1:1
- Совмещение:102 [Mate]: гайка T-паза m5_MIR_MIR1_MIR1:1 ↔ скоба_MIR1:1
- Совмещение:103 [Mate]: гайка T-паза m5_MIR_MIR1_MIR1:1 ↔ скоба_MIR1:1
- Угол:9 [Angle] (0 deg): гайка T-паза m5_MIR_MIR1_MIR1:2 ↔ скоба_MIR1:1
- Совмещение:104 [Mate]: гайка T-паза m5_MIR_MIR1_MIR1:2 ↔ скоба_MIR1:1
- Совмещение:105 [Mate]: гайка T-паза m5_MIR_MIR1_MIR1:2 ↔ скоба_MIR1:1
- Заподлицо:65 [Flush]: DIN 7991 M5x8:83 ↔ скоба_MIR1:1
- Заподлицо:66 [Flush]: DIN 7991 M5x8:84 ↔ скоба_MIR1:1
- Совмещение:108 [Mate]: скоба_MIR_MIR:1 ↔ гайка T-паза m5_MIR_MIR1_MIR_MIR:1
- Совмещение:109 [Mate]: скоба_MIR_MIR:1 ↔ гайка T-паза m5_MIR_MIR1_MIR_MIR:1
- Угол:10 [Angle] (0 deg): скоба_MIR_MIR:1 ↔ гайка T-паза m5_MIR_MIR1_MIR_MIR:1
- Совмещение:110 [Mate]: скоба_MIR_MIR:1 ↔ гайка T-паза m5_MIR_MIR1_MIR_MIR:2
- Совмещение:111 [Mate]: скоба_MIR_MIR:1 ↔ гайка T-паза m5_MIR_MIR1_MIR_MIR:2
- Угол:11 [Angle] (0 deg): скоба_MIR_MIR:1 ↔ гайка T-паза m5_MIR_MIR1_MIR_MIR:2
- Совмещение:112 [Mate]: скоба_MIR_MIR:1 ↔ DIN 7991 M5x8:85
- Заподлицо:67 [Flush]: скоба_MIR_MIR:1 ↔ DIN 7991 M5x8:85
- Заподлицо:68 [Flush]: скоба_MIR_MIR:1 ↔ DIN 7991 M5x8:86
- Совмещение:113 [Mate]: DIN 7991 M5x8:86 ↔ гайка T-паза m5_MIR_MIR1_MIR_MIR:2
- Заподлицо:69 [Flush] (130 mm): рама:1
- Совмещение:124 [Mate]: скоба_MIR1_MIR:1 ↔ гайка T-паза m5_MIR_MIR1_MIR1_MIR:2
- Совмещение:125 [Mate]: скоба_MIR1_MIR:1 ↔ гайка T-паза m5_MIR_MIR1_MIR1_MIR:2
- Угол:16 [Angle] (0 deg): скоба_MIR1_MIR:1 ↔ гайка T-паза m5_MIR_MIR1_MIR1_MIR:2
- Совмещение:126 [Mate]: скоба_MIR1_MIR:1 ↔ гайка T-паза m5_MIR_MIR1_MIR1_MIR:1
- Совмещение:127 [Mate]: скоба_MIR1_MIR:1 ↔ гайка T-паза m5_MIR_MIR1_MIR1_MIR:1
- Угол:17 [Angle] (0 deg): скоба_MIR1_MIR:1 ↔ гайка T-паза m5_MIR_MIR1_MIR1_MIR:1
- Заподлицо:74 [Flush]: скоба_MIR1_MIR:1 ↔ DIN 7991 M5x8:90
- Заподлицо:75 [Flush]: скоба_MIR1_MIR:1 ↔ DIN 7991 M5x8:89
- Угол:18 [Angle] (0 deg): гайка T-паза m5_MIR_MIR1_MIR_MIR_MIR:2 ↔ скоба_MIR_MIR_MIR:1
- Совмещение:128 [Mate]: гайка T-паза m5_MIR_MIR1_MIR_MIR_MIR:2 ↔ скоба_MIR_MIR_MIR:1
- Совмещение:129 [Mate]: гайка T-паза m5_MIR_MIR1_MIR_MIR_MIR:2 ↔ скоба_MIR_MIR_MIR:1
- Угол:19 [Angle] (0 deg): гайка T-паза m5_MIR_MIR1_MIR_MIR_MIR:1 ↔ скоба_MIR_MIR_MIR:1
- Совмещение:130 [Mate]: гайка T-паза m5_MIR_MIR1_MIR_MIR_MIR:1 ↔ скоба_MIR_MIR_MIR:1
- Совмещение:131 [Mate]: гайка T-паза m5_MIR_MIR1_MIR_MIR_MIR:1 ↔ скоба_MIR_MIR_MIR:1
- Заподлицо:76 [Flush]: скоба_MIR_MIR_MIR:1 ↔ DIN 7991 M5x8:88
- Совмещение:132 [Mate]: скоба_MIR_MIR_MIR:1 ↔ DIN 7991 M5x8:88
- Совмещение:133 [Mate]: гайка T-паза m5_MIR_MIR1_MIR_MIR_MIR:1 ↔ DIN 7991 M5x8:87
- Заподлицо:77 [Flush]: скоба_MIR_MIR_MIR:1 ↔ DIN 7991 M5x8:87
- Заподлицо:78 [Flush]: скоба_MIR_MIR_MIR_MIR:1 ↔ DIN 7991 M5x8:92
- Совмещение:134 [Mate]: скоба_MIR_MIR_MIR_MIR:1 ↔ DIN 7991 M5x8:91
- Заподлицо:79 [Flush]: скоба_MIR_MIR_MIR_MIR:1 ↔ DIN 7991 M5x8:91
- Совмещение:135 [Mate]: гайка T-паза m5_MIR_MIR1_MIR_MIR_MIR_MIR:1 ↔ DIN 7991 M5x8:92
- Совмещение:136 [Mate]: гайка T-паза m5_MIR_MIR1_MIR_MIR_MIR_MIR:1 ↔ скоба_MIR_MIR_MIR_MIR:1
- Совмещение:137 [Mate]: гайка T-паза m5_MIR_MIR1_MIR_MIR_MIR_MIR:1 ↔ скоба_MIR_MIR_MIR_MIR:1
- Угол:20 [Angle] (0 deg): гайка T-паза m5_MIR_MIR1_MIR_MIR_MIR_MIR:1 ↔ скоба_MIR_MIR_MIR_MIR:1
- Совмещение:138 [Mate]: гайка T-паза m5_MIR_MIR1_MIR_MIR_MIR_MIR:2 ↔ скоба_MIR_MIR_MIR_MIR:1
- Совмещение:139 [Mate]: гайка T-паза m5_MIR_MIR1_MIR_MIR_MIR_MIR:2 ↔ скоба_MIR_MIR_MIR_MIR:1
- Угол:21 [Angle] (0 deg): гайка T-паза m5_MIR_MIR1_MIR_MIR_MIR_MIR:2 ↔ скоба_MIR_MIR_MIR_MIR:1
- Заподлицо:80 [Flush]: скоба_MIR1_MIR_MIR:1 ↔ DIN 7991 M5x8:93
- Заподлицо:81 [Flush]: скоба_MIR1_MIR_MIR:1 ↔ DIN 7991 M5x8:94
- Угол:22 [Angle] (0 deg): скоба_MIR1_MIR_MIR:1 ↔ гайка T-паза m5_MIR_MIR1_MIR1_MIR_MIR:1
- Совмещение:140 [Mate]: скоба_MIR1_MIR_MIR:1 ↔ гайка T-паза m5_MIR_MIR1_MIR1_MIR_MIR:1
- Совмещение:141 [Mate]: скоба_MIR1_MIR_MIR:1 ↔ гайка T-паза m5_MIR_MIR1_MIR1_MIR_MIR:1
- Угол:23 [Angle] (0 deg): скоба_MIR1_MIR_MIR:1 ↔ гайка T-паза m5_MIR_MIR1_MIR1_MIR_MIR:2
- Совмещение:142 [Mate]: скоба_MIR1_MIR_MIR:1 ↔ гайка T-паза m5_MIR_MIR1_MIR1_MIR_MIR:2
- Совмещение:143 [Mate]: скоба_MIR1_MIR_MIR:1 ↔ гайка T-паза m5_MIR_MIR1_MIR1_MIR_MIR:2
- Угол:24 [Angle] (0 deg): скоба_MIR4:1 ↔ гайка T-паза m5_MIR_MIR1_MIR3:1
- Совмещение:144 [Mate]: скоба_MIR4:1 ↔ гайка T-паза m5_MIR_MIR1_MIR3:1
- Совмещение:145 [Mate]: скоба_MIR4:1 ↔ гайка T-паза m5_MIR_MIR1_MIR3:1
- Угол:25 [Angle] (0 deg): скоба_MIR4:1 ↔ гайка T-паза m5_MIR_MIR1_MIR3:2
- Совмещение:146 [Mate]: скоба_MIR4:1 ↔ гайка T-паза m5_MIR_MIR1_MIR3:2
- Совмещение:147 [Mate]: скоба_MIR4:1 ↔ гайка T-паза m5_MIR_MIR1_MIR3:2
- Заподлицо:82 [Flush]: скоба_MIR4:1 ↔ DIN 7991 M5x8:109
- Совмещение:148 [Mate]: скоба_MIR4:1 ↔ DIN 7991 M5x8:109
- Совмещение:149 [Mate]: гайка T-паза m5_MIR_MIR1_MIR3:2 ↔ DIN 7991 M5x8:110
- Заподлицо:83 [Flush]: скоба_MIR4:1 ↔ DIN 7991 M5x8:110
- Совмещение:150 [Mate]: гайка T-паза m5_MIR_MIR1_MIR_MIR2:2 ↔ скоба_MIR_MIR2:1
- Совмещение:151 [Mate]: гайка T-паза m5_MIR_MIR1_MIR_MIR2:2 ↔ скоба_MIR_MIR2:1
- Угол:26 [Angle] (0 deg): гайка T-паза m5_MIR_MIR1_MIR_MIR2:2 ↔ скоба_MIR_MIR2:1
- Совмещение:152 [Mate]: гайка T-паза m5_MIR_MIR1_MIR_MIR2:1 ↔ скоба_MIR_MIR2:1
- Совмещение:153 [Mate]: гайка T-паза m5_MIR_MIR1_MIR_MIR2:1 ↔ скоба_MIR_MIR2:1
- Угол:27 [Angle] (0 deg): гайка T-паза m5_MIR_MIR1_MIR_MIR2:1 ↔ скоба_MIR_MIR2:1
- Заподлицо:84 [Flush]: DIN 7991 M5x8:108 ↔ скоба_MIR_MIR2:1
- Заподлицо:85 [Flush]: DIN 7991 M5x8:107 ↔ скоба_MIR_MIR2:1
- Совмещение:154 [Mate]: гайка T-паза m5_MIR_MIR1_MIR1_MIR1:2 ↔ скоба_MIR1_MIR1:1
- Совмещение:155 [Mate]: гайка T-паза m5_MIR_MIR1_MIR1_MIR1:2 ↔ скоба_MIR1_MIR1:1
- Угол:28 [Angle] (0 deg): гайка T-паза m5_MIR_MIR1_MIR1_MIR1:2 ↔ скоба_MIR1_MIR1:1
- Совмещение:156 [Mate]: гайка T-паза m5_MIR_MIR1_MIR1_MIR1:1 ↔ скоба_MIR1_MIR1:1
- Совмещение:157 [Mate]: гайка T-паза m5_MIR_MIR1_MIR1_MIR1:1 ↔ скоба_MIR1_MIR1:1
- Угол:29 [Angle] (0 deg): гайка T-паза m5_MIR_MIR1_MIR1_MIR1:1 ↔ скоба_MIR1_MIR1:1
- Заподлицо:86 [Flush]: DIN 7991 M5x8:106 ↔ скоба_MIR1_MIR1:1
- Заподлицо:87 [Flush]: DIN 7991 M5x8:105 ↔ скоба_MIR1_MIR1:1
- Угол:30 [Angle] (0 deg): скоба_MIR_MIR_MIR1:1 ↔ гайка T-паза m5_MIR_MIR1_MIR_MIR_MIR1:2
- Совмещение:158 [Mate]: скоба_MIR_MIR_MIR1:1 ↔ гайка T-паза m5_MIR_MIR1_MIR_MIR_MIR1:2
- Совмещение:159 [Mate]: скоба_MIR_MIR_MIR1:1 ↔ гайка T-паза m5_MIR_MIR1_MIR_MIR_MIR1:2
- Угол:31 [Angle] (0 deg): скоба_MIR_MIR_MIR1:1 ↔ гайка T-паза m5_MIR_MIR1_MIR_MIR_MIR1:1
- Совмещение:160 [Mate]: скоба_MIR_MIR_MIR1:1 ↔ гайка T-паза m5_MIR_MIR1_MIR_MIR_MIR1:1
- Совмещение:161 [Mate]: скоба_MIR_MIR_MIR1:1 ↔ гайка T-паза m5_MIR_MIR1_MIR_MIR_MIR1:1
- Заподлицо:88 [Flush]: скоба_MIR_MIR_MIR1:1 ↔ DIN 7991 M5x8:104
- Совмещение:162 [Mate]: скоба_MIR_MIR_MIR1:1 ↔ DIN 7991 M5x8:104
- Совмещение:163 [Mate]: DIN 7991 M5x8:103 ↔ гайка T-паза m5_MIR_MIR1_MIR_MIR_MIR1:1
- Заподлицо:89 [Flush]: скоба_MIR_MIR_MIR1:1 ↔ DIN 7991 M5x8:103
- Заподлицо:90 [Flush]: скоба_MIR_MIR_MIR_MIR1:1 ↔ DIN 7991 M5x8:101
- Совмещение:164 [Mate]: скоба_MIR_MIR_MIR_MIR1:1 ↔ DIN 7991 M5x8:102
- Заподлицо:91 [Flush]: скоба_MIR_MIR_MIR_MIR1:1 ↔ DIN 7991 M5x8:102
- Совмещение:165 [Mate]: гайка T-паза m5_MIR_MIR1_MIR_MIR_MIR_MIR1:2 ↔ DIN 7991 M5x8:101
- Совмещение:166 [Mate]: гайка T-паза m5_MIR_MIR1_MIR_MIR_MIR_MIR1:2 ↔ скоба_MIR_MIR_MIR_MIR1:1
- Совмещение:167 [Mate]: гайка T-паза m5_MIR_MIR1_MIR_MIR_MIR_MIR1:2 ↔ скоба_MIR_MIR_MIR_MIR1:1
- Угол:32 [Angle] (0 deg): гайка T-паза m5_MIR_MIR1_MIR_MIR_MIR_MIR1:2 ↔ скоба_MIR_MIR_MIR_MIR1:1
- Совмещение:168 [Mate]: гайка T-паза m5_MIR_MIR1_MIR_MIR_MIR_MIR1:1 ↔ скоба_MIR_MIR_MIR_MIR1:1
- Совмещение:169 [Mate]: гайка T-паза m5_MIR_MIR1_MIR_MIR_MIR_MIR1:1 ↔ скоба_MIR_MIR_MIR_MIR1:1
- Угол:33 [Angle] (0 deg): гайка T-паза m5_MIR_MIR1_MIR_MIR_MIR_MIR1:1 ↔ скоба_MIR_MIR_MIR_MIR1:1
- Заподлицо:92 [Flush]: скоба_MIR1_MIR_MIR1:1 ↔ DIN 7991 M5x8:100
- Заподлицо:93 [Flush]: скоба_MIR1_MIR_MIR1:1 ↔ DIN 7991 M5x8:99
- Угол:34 [Angle] (0 deg): скоба_MIR1_MIR_MIR1:1 ↔ гайка T-паза m5_MIR_MIR1_MIR1_MIR_MIR1:2
- Совмещение:170 [Mate]: скоба_MIR1_MIR_MIR1:1 ↔ гайка T-паза m5_MIR_MIR1_MIR1_MIR_MIR1:2
- Совмещение:171 [Mate]: скоба_MIR1_MIR_MIR1:1 ↔ гайка T-паза m5_MIR_MIR1_MIR1_MIR_MIR1:2
- Угол:35 [Angle] (0 deg): скоба_MIR1_MIR_MIR1:1 ↔ гайка T-паза m5_MIR_MIR1_MIR1_MIR_MIR1:1
- Совмещение:172 [Mate]: скоба_MIR1_MIR_MIR1:1 ↔ гайка T-паза m5_MIR_MIR1_MIR1_MIR_MIR1:1
- Совмещение:173 [Mate]: скоба_MIR1_MIR_MIR1:1 ↔ гайка T-паза m5_MIR_MIR1_MIR1_MIR_MIR1:1
- Заподлицо:94 [Flush]: скоба_MIR_MIR_MIR_MIR_MIR:1 ↔ DIN 7991 M5x8:98
- Совмещение:174 [Mate]: скоба_MIR_MIR_MIR_MIR_MIR:1 ↔ DIN 7991 M5x8:98
- Заподлицо:95 [Flush]: скоба_MIR_MIR_MIR_MIR_MIR:1 ↔ DIN 7991 M5x8:97
- Угол:36 [Angle] (0 deg): гайка T-паза m5_MIR_MIR1_MIR_MIR_MIR_MIR_MIR:2 ↔ скоба_MIR_MIR_MIR_MIR_MIR:1
- Совмещение:175 [Mate]: гайка T-паза m5_MIR_MIR1_MIR_MIR_MIR_MIR_MIR:2 ↔ скоба_MIR_MIR_MIR_MIR_MIR:1
- Совмещение:176 [Mate]: гайка T-паза m5_MIR_MIR1_MIR_MIR_MIR_MIR_MIR:2 ↔ скоба_MIR_MIR_MIR_MIR_MIR:1
- Совмещение:177 [Mate]: гайка T-паза m5_MIR_MIR1_MIR_MIR_MIR_MIR_MIR:2 ↔ DIN 7991 M5x8:97
- Угол:37 [Angle] (0 deg): гайка T-паза m5_MIR_MIR1_MIR_MIR_MIR_MIR_MIR:1 ↔ скоба_MIR_MIR_MIR_MIR_MIR:1
- Совмещение:178 [Mate]: гайка T-паза m5_MIR_MIR1_MIR_MIR_MIR_MIR_MIR:1 ↔ скоба_MIR_MIR_MIR_MIR_MIR:1
- Совмещение:179 [Mate]: гайка T-паза m5_MIR_MIR1_MIR_MIR_MIR_MIR_MIR:1 ↔ скоба_MIR_MIR_MIR_MIR_MIR:1
- Совмещение:180 [Mate]: скоба_MIR1_MIR_MIR_MIR:1 ↔ гайка T-паза m5_MIR_MIR1_MIR1_MIR_MIR_MIR:1
- Совмещение:181 [Mate]: скоба_MIR1_MIR_MIR_MIR:1 ↔ гайка T-паза m5_MIR_MIR1_MIR1_MIR_MIR_MIR:1
- Угол:38 [Angle] (0 deg): скоба_MIR1_MIR_MIR_MIR:1 ↔ гайка T-паза m5_MIR_MIR1_MIR1_MIR_MIR_MIR:1
- Совмещение:182 [Mate]: скоба_MIR1_MIR_MIR_MIR:1 ↔ гайка T-паза m5_MIR_MIR1_MIR1_MIR_MIR_MIR:2
- Совмещение:183 [Mate]: скоба_MIR1_MIR_MIR_MIR:1 ↔ гайка T-паза m5_MIR_MIR1_MIR1_MIR_MIR_MIR:2
- Угол:39 [Angle] (0 deg): скоба_MIR1_MIR_MIR_MIR:1 ↔ гайка T-паза m5_MIR_MIR1_MIR1_MIR_MIR_MIR:2
- Заподлицо:96 [Flush]: скоба_MIR1_MIR_MIR_MIR:1 ↔ DIN 7991 M5x8:95
- Заподлицо:97 [Flush]: скоба_MIR1_MIR_MIR_MIR:1 ↔ DIN 7991 M5x8:96
